# Autodesk Inventor assembly: F_TOPO
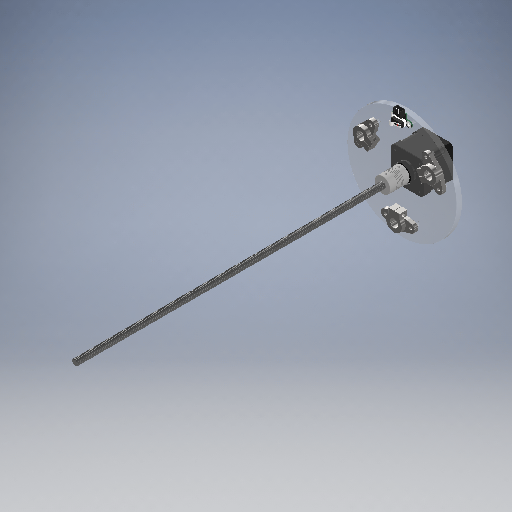
[picture p0: Inventor's stored thumbnail of the model, 512x512]
Saved by Autodesk Inventor 2025.1 (Build 291241020, 241B)
## iProperties
Created: 2025-05-02
Part Number: F_TOPO
Document SubType Name: Assembly
Designer: Nelson
Author: Nelson
## Documents named in this file (7)
- C:\Users\tiago\Documents\Inventor\SCRA\F_TOPO.iam
- C:\Users\tiago\Documents\Inventor\SCRA\Topo.ipt
- C:\Users\tiago\Documents\Inventor\SCRA\Lead screw 2pitch_8lead_400mm.ipt
- C:\Users\tiago\Documents\Inventor\SCRA\NEMA17 42-38.ipt
- C:\Users\tiago\Documents\Inventor\SCRA\shaft_coupler 5mm_to_8mm.ipt
- C:\Users\tiago\Documents\Inventor\SCRA\Linear_Shaft_Support_SHF10.ipt
- C:\Users\tiago\Documents\Inventor\SCRA\Limit_Switch.ipt
## Components (8 placed, 6 different names)
1. Topo:1 — Mate:1, Mate:2, Mate:3, Mate:4, Mate:5, Mate:6, Mate:7, Mate:8, Mate:9, Mate:10, Mate:11, Mate:12, Mate:17, Mate:18, Mate:19
2. Lead screw 2pitch_8lead_400mm:1 — Mate:13, Mate:14, Mate:16
3. NEMA17 42-38:1 — Mate:2, Mate:3, Mate:14, Mate:15, Mate:16
4. shaft_coupler 5mm_to_8mm:1 — Mate:13, Mate:15
5. Linear_Shaft_Support_SHF10:1 — Mate:4, Mate:9, Mate:10
6. Linear_Shaft_Support_SHF10:2 — Mate:5, Mate:7, Mate:12
7. Linear_Shaft_Support_SHF10:3 — Mate:6, Mate:8, Mate:11
8. Limit_Switch:1 — Mate:17, Mate:18, Mate:19
## Relationships (19: Mate 19)
- Mate:1: Topo:1
- Mate:2: Topo:1 ↔ NEMA17 42-38:1
- Mate:3: Topo:1 ↔ NEMA17 42-38:1
- Mate:4: Topo:1 ↔ Linear_Shaft_Support_SHF10:1
- Mate:5: Topo:1 ↔ Linear_Shaft_Support_SHF10:2
- Mate:6: Topo:1 ↔ Linear_Shaft_Support_SHF10:3
- Mate:7: Topo:1 ↔ Linear_Shaft_Support_SHF10:2
- Mate:8: Topo:1 ↔ Linear_Shaft_Support_SHF10:3
- Mate:9: Topo:1 ↔ Linear_Shaft_Support_SHF10:1
- Mate:10: Topo:1 ↔ Linear_Shaft_Support_SHF10:1
- Mate:11: Topo:1 ↔ Linear_Shaft_Support_SHF10:3
- Mate:12: Topo:1 ↔ Linear_Shaft_Support_SHF10:2
- Mate:13: Lead screw 2pitch_8lead_400mm:1 ↔ shaft_coupler 5mm_to_8mm:1
- Mate:14: Lead screw 2pitch_8lead_400mm:1 ↔ NEMA17 42-38:1
- Mate:15 (5 mm): NEMA17 42-38:1 ↔ shaft_coupler 5mm_to_8mm:1
- Mate:16 (1 mm): Lead screw 2pitch_8lead_400mm:1 ↔ NEMA17 42-38:1
- Mate:17: Topo:1 ↔ Limit_Switch:1
- Mate:18: Topo:1 ↔ Limit_Switch:1
- Mate:19: Topo:1 ↔ Limit_Switch:1
